# Autodesk Inventor assembly: DESENHO
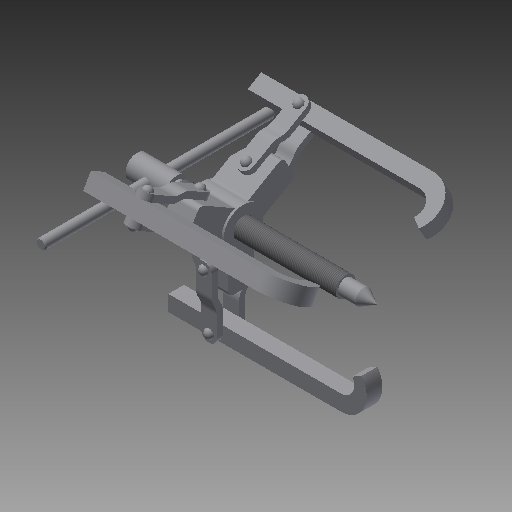
[picture p0: Inventor's stored thumbnail of the model, 512x512]
Saved by Autodesk Inventor 2017 (Build 210142000, 142)
## iProperties
Created: 2019-10-16
Part Number: DESENHO
Document SubType Name: Assembly
Designer: 20171enpro0154
Author: 20171enpro0154
## Documents named in this file (8)
- I:\DESENHO CONJUNTO\DESENHO.iam
- I:\DESENHO CONJUNTO\aranha.ipt
- I:\DESENHO CONJUNTO\parafuso.ipt
- I:\DESENHO CONJUNTO\manípulo.ipt
- I:\DESENHO CONJUNTO\rebite aranha.ipt
- I:\DESENHO CONJUNTO\jumelo.ipt
- I:\DESENHO CONJUNTO\rebite garra.ipt
- I:\DESENHO CONJUNTO\garra.ipt
## Components (18 placed, 7 different names)
1. aranha:1 — Mate:1, Mate:2, Mate:5, Insert:1, Angle:1
2. parafuso:1 — Mate:1, Mate:2, Mate:3, Mate:4, Mate:5
3. manípulo:1 — Mate:3, Mate:4
4. rebite aranha:1 — Insert:1, Insert:2, Insert:3
5. jumelo:1 — Insert:3, Mate:6, Insert:4
6. jumelo:2 — Insert:2, Angle:1, Mate:6, Insert:5
7. rebite garra:1 — Insert:4
8. garra:1 — Insert:5
9. rebite aranha:2
10. jumelo:3
11. jumelo:4
12. rebite garra:2
13. garra:2
14. rebite aranha:3
15. jumelo:5
16. jumelo:6
17. rebite garra:3
18. garra:3
## Component patterns: (3 elements, first: rebite aranha:1 + jumelo:1 + jumelo:2 + rebite garra:1 + garra:1)
## Relationships (12: Mate 6, Insert 5, Angle 1)
- Mate:1: aranha:1 ↔ parafuso:1
- Mate:2 (-25 mm): aranha:1 ↔ parafuso:1
- Mate:3: parafuso:1 ↔ manípulo:1
- Mate:4 (110 mm): parafuso:1 ↔ manípulo:1
- Mate:5: aranha:1 ↔ parafuso:1
- Insert:1 (6 mm): aranha:1 ↔ rebite aranha:1
- Insert:2: rebite aranha:1 ↔ jumelo:2
- Angle:1 (0 deg): aranha:1 ↔ jumelo:2
- Insert:3: rebite aranha:1 ↔ jumelo:1
- Mate:6: jumelo:1 ↔ jumelo:2
- Insert:4: jumelo:1 ↔ rebite garra:1
- Insert:5: jumelo:2 ↔ garra:1
